# Autodesk Inventor assembly: 4in Lazy Suzan
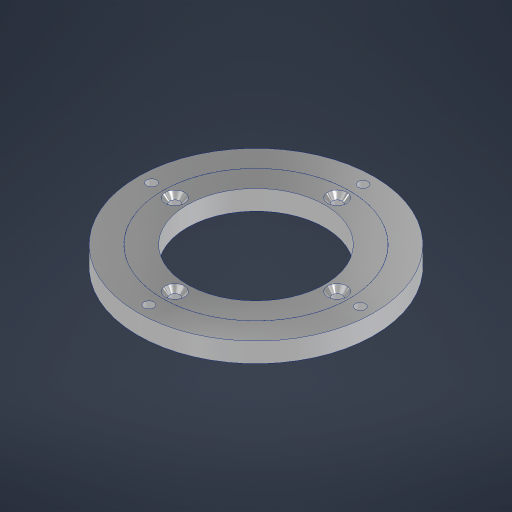
[picture p0: Inventor's stored thumbnail of the model, 512x512]
Saved by Autodesk Inventor 2023.4 (Build 274418000, 418)
## iProperties
Created: 2025-02-23
Part Number: 4in Lazy Suzan
Document SubType Name: Assembly
Designer: brand
Author: brand
## Documents named in this file (3)
- C:\Users\brand\OneDrive\Documents\GitHub\robotics 23\2025-ReefScape---CAD\COMMON PARTS\4in Lazy Suzan.iam
- C:\Users\brand\OneDrive\Documents\GitHub\robotics 23\2025-ReefScape---CAD\COMMON PARTS\4in LS-001.ipt
- C:\Users\brand\OneDrive\Documents\GitHub\robotics 23\2025-ReefScape---CAD\COMMON PARTS\4in LS-002.ipt
## Components (2 placed, 2 different names)
1. 4in LS-001:1 — Insert:1
2. 4in LS-002:1 — Insert:1
## Relationships (1: Insert 1)
- Insert:1: 4in LS-001:1 ↔ 4in LS-002:1
